# Autodesk Inventor assembly: Anglerfish_bonne_mamman_m12large_flipped_v0
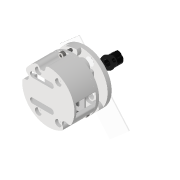
[picture p0: Inventor's stored thumbnail of the model, 180x180]
Saved by Autodesk Inventor 2022 (Build 260153000, 153)
## iProperties
Created: 2022-04-02
Part Number: Anglerfish_bonne_mamman_m12large_flipped_v0
Document SubType Name: Assembly
Designer: Prakash Lab
Author: Prakash Lab
## Documents named in this file (15)
- C:\Users\UC2\Documents\GitHub\Matchboxscope\INVENTOR\ANGLERFISH\Anglerfish_bonne_mamman_m12large_flipped_v0.iam
- C:\Users\UC2\Documents\GitHub\Matchboxscope\INVENTOR\ANGLERFISH\00_ESP3-CAM.iam
- C:\Users\UC2\Documents\GitHub\Matchboxscope\INVENTOR\ANGLERFISH\00_Powerbank.ipt
- C:\Users\UC2\Documents\GitHub\Matchboxscope\INVENTOR\ANGLERFISH\00_bonne_maman_jar.ipt
- C:\Users\UC2\Documents\GitHub\Matchboxscope\INVENTOR\ANGLERFISH\Matchboxscope_M12_Lensadapter_v0.ipt
- C:\Users\UC2\Documents\GitHub\Matchboxscope\INVENTOR\ANGLERFISH\00_toslink_launcher_v3.ipt
- C:\Users\UC2\Documents\GitHub\Matchboxscope\INVENTOR\ANGLERFISH\00_CCTV_M12_VCM_large.ipt
- C:\Users\UC2\Documents\GitHub\Matchboxscope\INVENTOR\ANGLERFISH\Anglerfish_flipped_LidMoun.ipt
- C:\Users\UC2\Documents\GitHub\Matchboxscope\INVENTOR\ANGLERFISH\Anglerfish_flipped_Baselayer.ipt
- C:\Users\UC2\Documents\GitHub\Matchboxscope\INVENTOR\ANGLERFISH\Anglerfish_flipped_Electronicsmount.ipt
- C:\Users\UC2\Documents\GitHub\Matchboxscope\INVENTOR\ANGLERFISH\00_Coverglass.ipt
- C:\Users\UC2\Documents\GitHub\Matchboxscope\INVENTOR\ANGLERFISH\00_Lid_Bonne_Mamman.ipt
- C:\Users\UC2\Documents\GitHub\Matchboxscope\INVENTOR\ANGLERFISH\Anglerfish_Lightplate_Tosslink_flipped.ipt
- C:\Users\UC2\Documents\GitHub\Matchboxscope\INVENTOR\ANGLERFISH\00_Magnet_8x3mm.ipt
- C:\Users\UC2\Documents\Inventor\Content Center Files\R2022\de-DE\DIN 912\DIN 912 - M3 x 0,5 x 12 x 10,75.ipt
## Components (24 placed, 14 different names)
1. 00_Powerbank:1
2. 00_toslink_launcher_v3:1 — Passend:28, Passend:29, Winkel:14
3. 00_bonne_maman_jar:1 — Passend:10, Winkel:1, Fluchtend:1
4. 00_ESP3-CAM:1 [sub-assembly] — Passend:23, Passend:24, Winkel:9, Winkel:11
5. 00_CCTV_M12_VCM_large:1 — Passend:30, Fluchtend:3, Einfügen:11
6. Matchboxscope_M12_Lensadapter_v0:1 — Einfügen:11
7. Anglerfish_flipped_Electronicsmount:1 — Einfügen:2, Winkel:11, Passend:30
8. Anglerfish_flipped_LidMoun:1 — Einfügen:3, Einfügen:5, Einfügen:6, Einfügen:7
9. Anglerfish_flipped_Baselayer:1 — Passend:23, Passend:24, Winkel:9, Einfügen:2, Winkel:10, Fluchtend:3, Einfügen:8, Einfügen:9, Einfügen:10, Einfügen:12, Einfügen:13, Einfügen:14, Einfügen:15, Einfügen:16, Einfügen:17
10. 00_Coverglass:1 — Passend:25, Passend:26, Winkel:13, Fluchtend:2
11. 00_Lid_Bonne_Mamman:1 — Einfügen:3, Winkel:12, Passend:25, Passend:26, Einfügen:4, Passend:27, Passend:29
12. Anglerfish_Lightplate_Tosslink_flipped:1 — Einfügen:4, Winkel:13, Passend:27, Fluchtend:2, Passend:28, Winkel:14
13. 00_Magnet_8x3mm:1 — Einfügen:7
14. 00_Magnet_8x3mm:2 — Einfügen:5
15. 00_Magnet_8x3mm:3 — Einfügen:9
16. 00_Magnet_8x3mm:4 — Einfügen:6
17. 00_Magnet_8x3mm:5 — Einfügen:8
18. 00_Magnet_8x3mm:6 — Einfügen:10
19. DIN 912 - ersetzt durch DIN EN ISO 4762 M3 x 12:1 — Einfügen:14
20. DIN 912 - ersetzt durch DIN EN ISO 4762 M3 x 12:2 — Einfügen:17
21. DIN 912 - ersetzt durch DIN EN ISO 4762 M3 x 12:4 — Einfügen:15
22. DIN 912 - ersetzt durch DIN EN ISO 4762 M3 x 12:5 — Einfügen:12
23. DIN 912 - ersetzt durch DIN EN ISO 4762 M3 x 12:6 — Einfügen:16
24. DIN 912 - ersetzt durch DIN EN ISO 4762 M3 x 12:7 — Einfügen:13
## Relationships (36: Insert 16, Mate 9, Angle 8, Flush 3)
- Passend:10 [Mate]: 00_bonne_maman_jar:1
- Winkel:1 [Angle] (0 deg): 00_bonne_maman_jar:1
- Fluchtend:1 [Flush]: 00_bonne_maman_jar:1
- [Angle] (45 deg): Anglerfish_flipped_Electronicsmount:1 ↔ Anglerfish_flipped_LidMoun:1
- Passend:23 [Mate]: 00_ESP3-CAM:1 ↔ Anglerfish_flipped_Baselayer:1
- Passend:24 [Mate]: 00_ESP3-CAM:1 ↔ Anglerfish_flipped_Baselayer:1
- Winkel:9 [Angle] (180 deg): 00_ESP3-CAM:1 ↔ Anglerfish_flipped_Baselayer:1
- Einfügen:2 [Insert]: Anglerfish_flipped_Electronicsmount:1 ↔ Anglerfish_flipped_Baselayer:1
- Winkel:10 [Angle] (180 deg): Anglerfish_flipped_Baselayer:1
- Winkel:11 [Angle] (180 deg): 00_ESP3-CAM:1 ↔ Anglerfish_flipped_Electronicsmount:1
- Einfügen:3 [Insert]: Anglerfish_flipped_LidMoun:1 ↔ 00_Lid_Bonne_Mamman:1
- Winkel:12 [Angle] (0 deg): 00_Lid_Bonne_Mamman:1
- Passend:25 [Mate]: 00_Coverglass:1 ↔ 00_Lid_Bonne_Mamman:1
- Passend:26 [Mate]: 00_Coverglass:1 ↔ 00_Lid_Bonne_Mamman:1
- Einfügen:4 [Insert] (1 mm): 00_Lid_Bonne_Mamman:1 ↔ Anglerfish_Lightplate_Tosslink_flipped:1
- Winkel:13 [Angle] (180 deg): 00_Coverglass:1 ↔ Anglerfish_Lightplate_Tosslink_flipped:1
- Passend:27 [Mate]: 00_Lid_Bonne_Mamman:1 ↔ Anglerfish_Lightplate_Tosslink_flipped:1
- Fluchtend:2 [Flush]: 00_Coverglass:1 ↔ Anglerfish_Lightplate_Tosslink_flipped:1
- Passend:28 [Mate]: 00_toslink_launcher_v3:1 ↔ Anglerfish_Lightplate_Tosslink_flipped:1
- Passend:29 [Mate]: 00_toslink_launcher_v3:1 ↔ 00_Lid_Bonne_Mamman:1
- Winkel:14 [Angle] (0 deg): 00_toslink_launcher_v3:1 ↔ Anglerfish_Lightplate_Tosslink_flipped:1
- Passend:30 [Mate]: 00_CCTV_M12_VCM_large:1 ↔ Anglerfish_flipped_Electronicsmount:1
- Fluchtend:3 [Flush]: 00_CCTV_M12_VCM_large:1 ↔ Anglerfish_flipped_Baselayer:1
- Einfügen:5 [Insert]: Anglerfish_flipped_LidMoun:1 ↔ 00_Magnet_8x3mm:2
- Einfügen:6 [Insert]: Anglerfish_flipped_LidMoun:1 ↔ 00_Magnet_8x3mm:4
- Einfügen:7 [Insert]: Anglerfish_flipped_LidMoun:1 ↔ 00_Magnet_8x3mm:1
- Einfügen:8 [Insert]: Anglerfish_flipped_Baselayer:1 ↔ 00_Magnet_8x3mm:5
- Einfügen:9 [Insert]: Anglerfish_flipped_Baselayer:1 ↔ 00_Magnet_8x3mm:3
- Einfügen:10 [Insert]: Anglerfish_flipped_Baselayer:1 ↔ 00_Magnet_8x3mm:6
- Einfügen:11 [Insert]: 00_CCTV_M12_VCM_large:1 ↔ Matchboxscope_M12_Lensadapter_v0:1
- Einfügen:12 [Insert]: Anglerfish_flipped_Baselayer:1 ↔ DIN 912 - ersetzt durch DIN EN ISO 4762 M3 x 12:5
- Einfügen:13 [Insert]: Anglerfish_flipped_Baselayer:1 ↔ DIN 912 - ersetzt durch DIN EN ISO 4762 M3 x 12:7
- Einfügen:14 [Insert]: Anglerfish_flipped_Baselayer:1 ↔ DIN 912 - ersetzt durch DIN EN ISO 4762 M3 x 12:1
- Einfügen:15 [Insert]: Anglerfish_flipped_Baselayer:1 ↔ DIN 912 - ersetzt durch DIN EN ISO 4762 M3 x 12:4
- Einfügen:16 [Insert]: Anglerfish_flipped_Baselayer:1 ↔ DIN 912 - ersetzt durch DIN EN ISO 4762 M3 x 12:6
- Einfügen:17 [Insert]: Anglerfish_flipped_Baselayer:1 ↔ DIN 912 - ersetzt durch DIN EN ISO 4762 M3 x 12:2
